# Autodesk Inventor assembly: FreeBOT_mech_v2
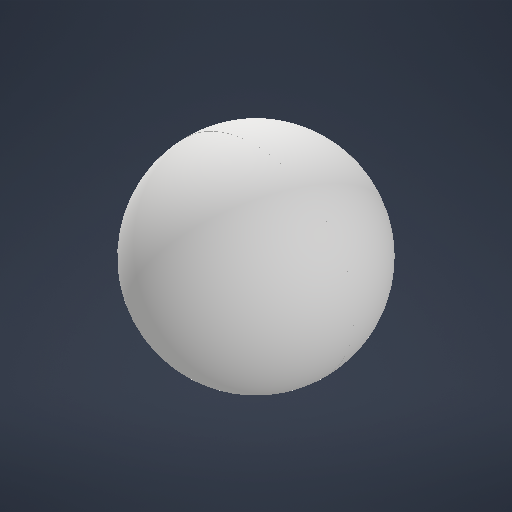
[picture p0: Inventor's stored thumbnail of the model, 512x512]
Saved by Autodesk Inventor 2027 (Build 310192060, 192F)
## iProperties
Created: 1601-01-02
Part Number: FreeBOT_mech_v2
Document SubType Name: Assembly
Designer: loren
Part Number: GM12-N20VA-Motor
Sending System: SOLIDWORKS 2018
Last Saved Date: 2022-07-07
Author: loren
## Documents named in this file (25)
- C:\Users\loren\Desktop\Tesi Magistrale\CAD\FreeBOT\FreeBOT_mech_v2.iam
- C:\Users\loren\Downloads\n20-14.snapshot.1\N20后侧输出轴\GM12-N20VA-Motor\M057-8Y01A.iam
- C:\Users\loren\Downloads\n20-14.snapshot.1\N20后侧输出轴\GM12-N20VA-Motor\减速机支架.ipt
- C:\Users\loren\Downloads\n20-14.snapshot.1\N20后侧输出轴\GM12-N20VA-Motor\十字沉头螺丝.ipt
- C:\Users\loren\Downloads\n20-14.snapshot.1\N20后侧输出轴\GM12-N20VA-Motor\Engrenagem reta21-15.ipt
- C:\Users\loren\Downloads\n20-14.snapshot.1\N20后侧输出轴\GM12-N20VA-Motor\Engrenagem reta27-18.ipt
- C:\Users\loren\Downloads\n20-14.snapshot.1\N20后侧输出轴\GM12-N20VA-Motor\Engrenagem reta28-D.ipt
- C:\Users\loren\Downloads\n20-14.snapshot.1\N20后侧输出轴\GM12-N20VA-Motor\Engrenagem reta25-17.ipt
- C:\Users\loren\Downloads\n20-14.snapshot.1\N20后侧输出轴\GM12-N20VA-Motor\Engrenagem reta12.ipt
- C:\Users\loren\Downloads\n20-14.snapshot.1\N20后侧输出轴\GM12-N20VA-Motor\Engrenagem reta22-11.ipt
- C:\Users\loren\Desktop\Tesi Magistrale\CAD\FreeBOT\chassis.ipt
- C:\Users\loren\Desktop\Tesi Magistrale\CAD\FreeBOT\chassis3.ipt
- C:\Users\loren\Desktop\Tesi Magistrale\CAD\FreeBOT\Pololu-Wheel-32x7mm.iam
- C:\Users\loren\Desktop\Tesi Magistrale\CAD\FreeBOT\tronco_ruote.ipt
- C:\Users\loren\Desktop\Tesi Magistrale\CAD\FreeBOT\tronco_ruota_2.ipt
- C:\Users\loren\Desktop\Tesi Magistrale\CAD\FreeBOT\chassis 2.ipt
- C:\Users\loren\Desktop\Tesi Magistrale\CAD\FreeBOT\tronco_ruota3.ipt
- C:\Users\loren\Desktop\Tesi Magistrale\CAD\FreeBOT\magnete.ipt
- C:\Users\loren\Desktop\Tesi Magistrale\CAD\FreeBOT\guscio sferico B.ipt.iam
- C:\Users\loren\Downloads\pololu-ball-caster-with-3-8-plastic-metal-ball-1.snapshot.3\Rueda loca\Pololu Ball Caster\base.ipt
- C:\Users\loren\Downloads\pololu-ball-caster-with-3-8-plastic-metal-ball-1.snapshot.3\Rueda loca\Pololu Ball Caster\ball.ipt
- C:\Users\loren\Desktop\Tesi Magistrale\CAD\FreeBOT\telaio per casters.ipt
- C:\Users\loren\Desktop\Tesi Magistrale\CAD\FreeBOT\base_telaio_casters.ipt
- C:\Users\loren\Desktop\Tesi Magistrale\CAD\FreeBOT\guscio sferico_A.iam
- guscio sferico B.ipt
## Components (47 placed, 34 different names)
1. M057-8Y01A-1 [sub-assembly] — Rigid:1, Rotational:1, Mate:4, Mate:5, Mate:6
2. 减速机支架-1 — Rigid:1, Rigid:2, Rigid:3, Rotational:2, Rotational:3, Rotational:4, Rotational:5, Rotational:6, Rotational:7, Mate:7, Mate:13
3. 十字沉头螺丝-1 — Rigid:3
4. 十字沉头螺丝-2 — Rigid:2
5. Engrenagem reta21-15-1 — Rotational:4
6. Engrenagem reta27-18-1 — Rotational:6
7. Engrenagem reta28-D-1 — Rotational:7, Mate:15, Rigid:7
8. Engrenagem reta25-17-1 — Rotational:5
9. Engrenagem reta12-1 — Rotational:1
10. Engrenagem reta22-11-1 — Rotational:2
11. Engrenagem reta21-15-2 — Rotational:3
12. chassis:1 — Mate:1, Mate:2, Mate:3, Mate:4, Mate:5, Mate:8, Mate:9, Mate:10, Mate:11, Rigid:19, Rigid:26, Rigid:27, Rigid:28, Rigid:29
13. chassis3:1 — Mate:1, Mate:2, Mate:3, Mate:6, Mate:7, Mate:13
14. M057-8Y01A:2 [sub-assembly] — Mate:10, Mate:11, Mate:12
15. 减速机支架:2 — Mate:14
16. 十字沉头螺丝:3
17. 十字沉头螺丝:4
18. Engrenagem reta21-15:3
19. Engrenagem reta27-18:2
20. Engrenagem reta28-D:2 — Mate:16, Rigid:25
21. Engrenagem reta25-17:2
22. Engrenagem reta12:2
23. Engrenagem reta22-11:2
24. Engrenagem reta21-15:4
25. chassis3:2 — Mate:8, Mate:9, Mate:12, Mate:14
26. Pololu-Wheel-32x7mm:1 [sub-assembly] — Rigid:17, Rigid:18
27. tronco_ruote:1 — Mate:15, Rigid:7, Rigid:16
28. tronco_ruota_2:1 — Rigid:16, Rigid:17
29. tronco_ruota_2:2 — Rigid:18
30. chassis 2:1 — Rigid:19, Rigid:20
31. tronco_ruota3:1 — Rigid:20
32. Pololu-Wheel-32x7mm:2 [sub-assembly]
33. tronco_ruote:2 — Mate:16, Rigid:25
34. tronco_ruota_2:3
35. tronco_ruota_2:4
36. chassis 2:2 — Rigid:26
37. tronco_ruota3:2
38. magnete:1 — Rigid:27
39. guscio sferico B.ipt:1 [sub-assembly] — Mate:18
40. base:1 — Ball:1, Rotational:15, Rotational:16
41. ball:1 — Ball:1
42. telaio per casters:1 — Rotational:15, Rotational:16, Mate:17, Rotational:17, Rotational:18, Rotational:19, Rotational:20, Rigid:30
43. base:2 — Mate:17, Rotational:17, Rotational:18, Rotational:19, Rotational:20
44. ball:2
45. base_telaio_casters:1 — Rigid:28
46. base_telaio_casters:2 — Rigid:29, Rigid:30
47. guscio sferico_A:1 [sub-assembly] — Mate:18
## Relationships (62: WeldJoint 22, RevoluteJoint 20, Mate 18, BallJoint 2)
- Rigid:1 [WeldJoint]: M057-8Y01A-1 ↔ 减速机支架-1
- Rigid:2 [WeldJoint]: 减速机支架-1 ↔ 十字沉头螺丝-2
- Rigid:3 [WeldJoint]: 减速机支架-1 ↔ 十字沉头螺丝-1
- Rotational:1 [RevoluteJoint]: M057-8Y01A-1 ↔ Engrenagem reta12-1
- Rotational:2 [RevoluteJoint]: 减速机支架-1 ↔ Engrenagem reta22-11-1
- Rotational:3 [RevoluteJoint]: 减速机支架-1 ↔ Engrenagem reta21-15-2
- Rotational:4 [RevoluteJoint]: 减速机支架-1 ↔ Engrenagem reta21-15-1
- Rotational:5 [RevoluteJoint]: 减速机支架-1 ↔ Engrenagem reta25-17-1
- Rotational:6 [RevoluteJoint]: 减速机支架-1 ↔ Engrenagem reta27-18-1
- Rotational:7 [RevoluteJoint]: 减速机支架-1 ↔ Engrenagem reta28-D-1
- Mate:1: chassis:1 ↔ chassis3:1
- Mate:2: chassis:1 ↔ chassis3:1
- Mate:3: chassis:1 ↔ chassis3:1
- Mate:4: M057-8Y01A-1 ↔ chassis:1
- Mate:5: M057-8Y01A-1 ↔ chassis:1
- Mate:6: M057-8Y01A-1 ↔ chassis3:1
- Mate:7: 减速机支架-1 ↔ chassis3:1
- [WeldJoint]: M057-8Y01A:2 ↔ 减速机支架:2
- [WeldJoint]: 减速机支架:2 ↔ 十字沉头螺丝:4
- [WeldJoint]: 减速机支架:2 ↔ 十字沉头螺丝:3
- [RevoluteJoint]: M057-8Y01A:2 ↔ Engrenagem reta12:2
- [RevoluteJoint]: 减速机支架:2 ↔ Engrenagem reta22-11:2
- [RevoluteJoint]: 减速机支架:2 ↔ Engrenagem reta21-15:4
- [RevoluteJoint]: 减速机支架:2 ↔ Engrenagem reta21-15:3
- [RevoluteJoint]: 减速机支架:2 ↔ Engrenagem reta25-17:2
- [RevoluteJoint]: 减速机支架:2 ↔ Engrenagem reta27-18:2
- [RevoluteJoint]: 减速机支架:2 ↔ Engrenagem reta28-D:2
- Mate:8: chassis:1 ↔ chassis3:2
- Mate:9: chassis:1 ↔ chassis3:2
- Mate:10: chassis:1 ↔ M057-8Y01A:2
- Mate:11: chassis:1 ↔ M057-8Y01A:2
- Mate:12: M057-8Y01A:2 ↔ chassis3:2
- Mate:13: 减速机支架-1 ↔ chassis3:1
- Mate:14: 减速机支架:2 ↔ chassis3:2
- Mate:15: Engrenagem reta28-D-1 ↔ tronco_ruote:1
- Rigid:7 [WeldJoint]: Engrenagem reta28-D-1 ↔ tronco_ruote:1
- Rigid:16 [WeldJoint]: tronco_ruote:1 ↔ tronco_ruota_2:1
- Rigid:17 [WeldJoint]: Pololu-Wheel-32x7mm:1 ↔ tronco_ruota_2:1
- Rigid:18 [WeldJoint]: Pololu-Wheel-32x7mm:1 ↔ tronco_ruota_2:2
- Rigid:19 [WeldJoint]: chassis:1 ↔ chassis 2:1
- Rigid:20 [WeldJoint]: chassis 2:1 ↔ tronco_ruota3:1
- [WeldJoint]: tronco_ruote:2 ↔ tronco_ruota_2:3
- [WeldJoint]: Pololu-Wheel-32x7mm:2 ↔ tronco_ruota_2:3
- [WeldJoint]: Pololu-Wheel-32x7mm:2 ↔ tronco_ruota_2:4
- [WeldJoint]: chassis 2:2 ↔ tronco_ruota3:2
- Mate:16: Engrenagem reta28-D:2 ↔ tronco_ruote:2
- Rigid:25 [WeldJoint]: Engrenagem reta28-D:2 ↔ tronco_ruote:2
- Rigid:26 [WeldJoint]: chassis:1 ↔ chassis 2:2
- Rigid:27 [WeldJoint]: chassis:1 ↔ magnete:1
- Ball:1: base:1 ↔ ball:1
- Rotational:15 [RevoluteJoint]: base:1 ↔ telaio per casters:1
- Rotational:16 [RevoluteJoint]: base:1 ↔ telaio per casters:1
- [BallJoint]: base:2 ↔ ball:2
- Mate:17: telaio per casters:1 ↔ base:2
- Rotational:17 [RevoluteJoint]: telaio per casters:1 ↔ base:2
- Rotational:18 [RevoluteJoint]: telaio per casters:1 ↔ base:2
- Rotational:19 [RevoluteJoint]: telaio per casters:1 ↔ base:2
- Rotational:20 [RevoluteJoint]: telaio per casters:1 ↔ base:2
- Rigid:28 [WeldJoint]: chassis:1 ↔ base_telaio_casters:1
- Rigid:29 [WeldJoint]: chassis:1 ↔ base_telaio_casters:2
- Rigid:30 [WeldJoint]: telaio per casters:1 ↔ base_telaio_casters:2
- Mate:18: guscio sferico B.ipt:1 ↔ guscio sferico_A:1
## Named parameters: d38_d0 = 0 mm, d39_d1 = 0 mm, d40_d2 = 0 mm, d41_d3 = 0 mm, d42_d4 = -49.508001 deg, d43_d7 = 0 mm, d44_d8 = -10.647068 deg, d45_d11 = 0 mm, d46_d12 = -35.599622 deg, d47_d15 = 0 mm, d48_d16 = 0.019573 deg, d49_d19 = 0 mm, d50_d20 = 17.369695 deg, d51_d23 = 0 mm, d52_d24 = -11.795615 deg, d53_d27 = 0 mm, d54_d28 = 5.187892 deg, d76_d75 = 0 mm, d77_d66 = 0 mm, d78_d67 = 7.193377 deg, d79_d70 = 0 mm, d80_d71 = 0 mm
